# Autodesk Inventor assembly: PistonWorkHeadMini
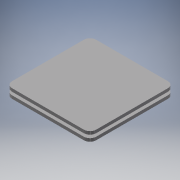
[picture p0: Inventor's stored thumbnail of the model, 180x180]
Saved by Autodesk Inventor 2016 (Build 200138000, 138)
## iProperties
Created: 2015-08-02
Part Number: PistonWorkHeadMini
Document SubType Name: Assembly
Designer: myhome
Author: myhome
## Documents named in this file (3)
- C:\Users\myhome\Documents\Inventor\Printer\PistonHead\PistonWorkHeadMini.iam
- C:\Users\myhome\Documents\Inventor\Printer\PistonHead\PistonWorkHeadInnerMini.ipt
- C:\Users\myhome\Documents\Inventor\Printer\PistonHead\PistonWorkHeadMini.ipt
## Components (3 placed, 2 different names)
1. PistonFeederHeadInnerMini:1 — Rigid:1, Rigid:2
2. PistonFeederHeadMini:1 — Rigid:2
3. PistonFeederHeadMini:2 — Rigid:1
## Relationships (2: WeldJoint 2)
- Rigid:1 [WeldJoint]: PistonFeederHeadInnerMini:1 ↔ PistonFeederHeadMini:2
- Rigid:2 [WeldJoint]: PistonFeederHeadInnerMini:1 ↔ PistonFeederHeadMini:1
